# Autodesk Inventor assembly: Top Lithium Modules
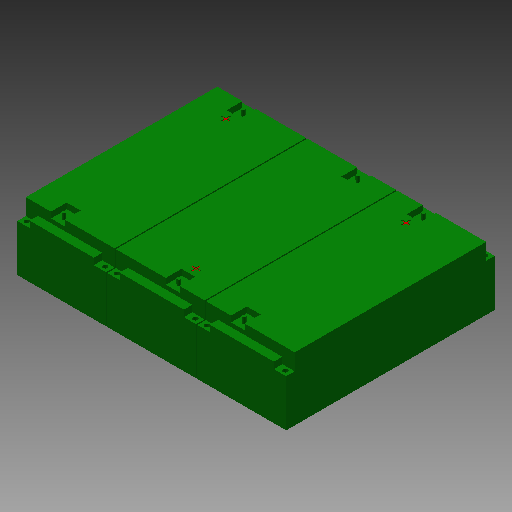
[picture p0: Inventor's stored thumbnail of the model, 512x512]
Saved by Autodesk Inventor 2017 (Build 210142000, 142)
## iProperties
Created: 2022-08-15
Part Number: Top Lithium Modules
Document SubType Name: Assembly
Designer: JTS
Author: JTS
## Documents named in this file (2)
- C:\Users\Windermac\Desktop\MASTER Honda Insight G1 IMA Bay\Top Lithium Modules.iam
- C:\Users\Windermac\Desktop\MASTER Honda Insight G1 IMA Bay\47Ah-FoMoCo.ipt
## Components (3 placed, 1 different names)
1. 47Ah-FoMoCo:1 — Flush:2, Mate:1, Mate:2, Flush:3, Flush:4
2. 47Ah-FoMoCo:2 — Flush:1, Flush:2, Mate:1, Flush:4
3. 47Ah-FoMoCo:3 — Flush:1, Mate:2, Flush:3
## Relationships (6: Flush 4, Mate 2)
- Flush:1: 47Ah-FoMoCo:2 ↔ 47Ah-FoMoCo:3
- Flush:2: 47Ah-FoMoCo:1 ↔ 47Ah-FoMoCo:2
- Mate:1 (2 mm): 47Ah-FoMoCo:1 ↔ 47Ah-FoMoCo:2
- Mate:2 (2 mm): 47Ah-FoMoCo:1 ↔ 47Ah-FoMoCo:3
- Flush:3: 47Ah-FoMoCo:1 ↔ 47Ah-FoMoCo:3
- Flush:4: 47Ah-FoMoCo:1 ↔ 47Ah-FoMoCo:2
